# Autodesk Inventor assembly: snap-enclosure
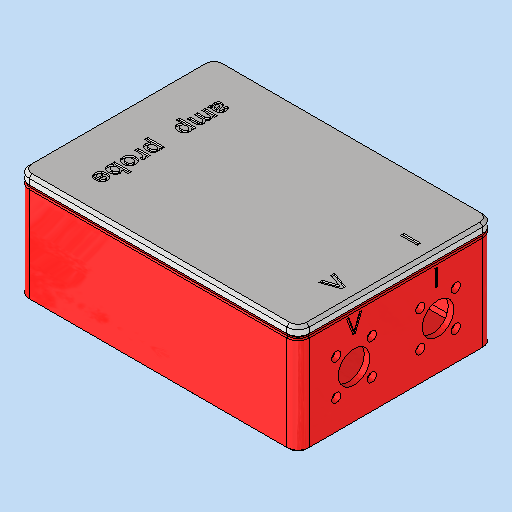
[picture p0: Inventor's stored thumbnail of the model, 512x512]
Saved by Autodesk Inventor 2025 (Build 290162000, 162)
## iProperties
Created: 2025-01-28
Part Number: snap-enclosure
Document SubType Name: Assembly
Designer: queezz
Author: queezz
## Documents named in this file (3)
- C:\Users\queez\Dropbox\Drawings\PIHTI\ElectronicsBox\snap-enclosure.iam
- C:\Users\queez\Dropbox\Drawings\PIHTI\ElectronicsBox\lp-box-snap.ipt
- C:\Users\queez\Dropbox\Drawings\PIHTI\ElectronicsBox\lid-snap.ipt
## Components (2 placed, 2 different names)
1. lp-box-snap:1 — Rigid:1
2. lid-snap:1 — Rigid:1
## Relationships (1: WeldJoint 1)
- Rigid:1 [WeldJoint]: lp-box-snap:1 ↔ lid-snap:1
